# Autodesk Inventor assembly: Mousetrap
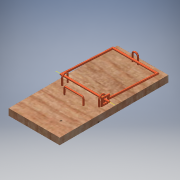
[picture p0: Inventor's stored thumbnail of the model, 180x180]
Saved by Autodesk Inventor 2016 (Build 200138000, 138)
## iProperties
Created: 2017-11-16
Part Number: Mousetrap
Document SubType Name: Assembly
Designer: shen95841
Author: shen95841
## Documents named in this file (5)
- E:\IED7_ShenF\IED7_Shen\IED7_Mousetrap\P3.5_Shen_Mousetrap\Mousetrap.iam
- E:\IED7_ShenF\IED7_Shen\IED7_Mousetrap\P3.5_Shen_Mousetrap\Mousetrap_Base.ipt
- E:\IED7_ShenF\IED7_Shen\IED7_Mousetrap\P3.5_Shen_Mousetrap\Small_Staple.ipt
- E:\IED7_ShenF\IED7_Shen\IED7_Mousetrap\P3.5_Shen_Mousetrap\Large_Staple.ipt
- E:\IED7_ShenF\IED7_Shen\IED7_Mousetrap\P3.5_Shen_Mousetrap\Hammer.ipt
## Components (6 placed, 4 different names)
1. Mousetrap_Base:1 — Insert:1, Insert:2, Insert:3, Insert:4, Insert:5, Insert:6, Insert:7, Insert:8
2. Small_Staple:1 — Insert:1, Insert:2
3. Small_Staple:2 — Insert:3, Insert:4, Mate:1
4. Small_Staple:3 — Insert:5, Insert:6, Mate:2
5. Large_Staple:1 — Insert:7, Insert:8
6. Hammer:1 — Mate:5
## Relationships (13: Insert 8, Mate 5)
- Insert:1: Mousetrap_Base:1 ↔ Small_Staple:1
- Insert:2: Mousetrap_Base:1 ↔ Small_Staple:1
- Insert:3: Mousetrap_Base:1 ↔ Small_Staple:2
- Insert:4: Mousetrap_Base:1 ↔ Small_Staple:2
- Insert:5: Mousetrap_Base:1 ↔ Small_Staple:3
- Insert:6: Mousetrap_Base:1 ↔ Small_Staple:3
- Insert:7: Mousetrap_Base:1 ↔ Large_Staple:1
- Insert:8: Mousetrap_Base:1 ↔ Large_Staple:1
- Mate:1: Small_Staple:2
- Mate:2: Small_Staple:3
- Mate:3
- Mate:4
- Mate:5: Hammer:1
